# Autodesk Inventor assembly: arduino_box
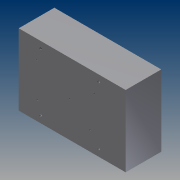
[picture p0: Inventor's stored thumbnail of the model, 180x180]
Saved by Autodesk Inventor 2011 SP1 (Build 150282100, 282)
## iProperties
Created: 2011-12-13
Part Number: arduino_box
Document SubType Name: Assembly
Designer: Nathan
Author: Nathan
## Documents named in this file (3)
- C:\Users\Nathan\Documents\Inventor\Quadcopter\arduino_box.iam
- C:\Users\Nathan\Documents\Inventor\Quadcopter\project box.ipt
- C:\Users\Nathan\Documents\Inventor\Quadcopter\Imported Components\User Library-Arduino Mega\Assembly2.iam
## Components (2 placed, 2 different names)
1. project box:1 — Mate:1, Angle:1, Mate:2
2. Assembly2:1 [sub-assembly] — Mate:1, Angle:1, Mate:2
## Relationships (3: Mate 2, Angle 1)
- Mate:1: project box:1 ↔ Assembly2:1
- Angle:1 (0 deg): project box:1 ↔ Assembly2:1
- Mate:2 (7.9375 mm): project box:1 ↔ Assembly2:1
